# Autodesk Inventor assembly: ròng rọc
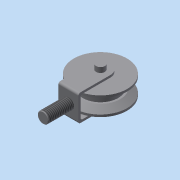
[picture p0: Inventor's stored thumbnail of the model, 180x180]
Saved by Autodesk Inventor 2018 (Build 220112000, 112)
## iProperties
Created: 2020-08-11
Part Number: ròng rọc
Document SubType Name: Assembly
Designer: ASUS
Author: ASUS
## Documents named in this file (3)
- E:\CTU\Skylight\Bản vẽ\Bản vẽ 3D\ròng rọc\ròng rọc.iam
- E:\CTU\Skylight\Bản vẽ\Bản vẽ 3D\ròng rọc\Giá đỡ ròng rọc.ipt
- E:\CTU\Skylight\Bản vẽ\Bản vẽ 3D\ròng rọc\Ròng rọc 48mm.ipt
## Components (2 placed, 2 different names)
1. Giá đỡ ròng rọc:1 — Mate:1, Flush:1
2. Ròng rọc 48mm:1 — Mate:1, Flush:1
## Relationships (2: Mate 1, Flush 1)
- Mate:1: Giá đỡ ròng rọc:1 ↔ Ròng rọc 48mm:1
- Flush:1 (3.5 mm): Giá đỡ ròng rọc:1 ↔ Ròng rọc 48mm:1
